# Autodesk Inventor assembly: MIR_Tower Pro 9g Micro Servo SG901
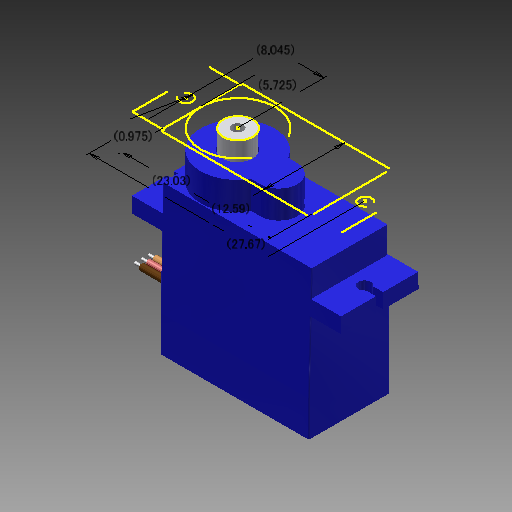
[picture p0: Inventor's stored thumbnail of the model, 512x512]
Saved by Autodesk Inventor 2018.1 (Build 221171000, 171)
## iProperties
Created: 2015-05-27
Part Number: MIR_Tower Pro 9g Micro Servo SG901
Material: 一般
Document SubType Name: Assembly
Designer: sktom
Author: sktom
Sending System: SolidWorks 2014
Last Author: Simon
Last Saved: 2015-06-03
## Documents named in this file (3)
- D:\CloudStrage\OneDrive\CAD\MAJ\hackberry\HACKberry-hardware\3D_69%inlength\Inventor\HbHandForChild\servo\MIR_Tower Pro 9g Micro Servo SG901.iam
- D:\CloudStrage\OneDrive\CAD\MAJ\hackberry\HACKberry-hardware\3D_69%inlength\Inventor\HbHandForChild\servo\MIR_Tower Pro 9g Micro Servo SG901.ipt
- D:\CloudStrage\OneDrive\CAD\MAJ\hackberry\HACKberry-hardware\3D_69%inlength\Inventor\HbHandForChild\servo\MIR_SG90 plastic Horn1.ipt
## Components (2 placed, 2 different names)
1. MIR_Tower Pro 9g Micro Servo SG901:1 — 挿入:1
2. MIR_SG90 plastic Horn1:1 — 挿入:1
## Relationships (1: Insert 1)
- 挿入:1 [Insert]: MIR_Tower Pro 9g Micro Servo SG901:1 ↔ MIR_SG90 plastic Horn1:1
